# Autodesk Inventor assembly: keel
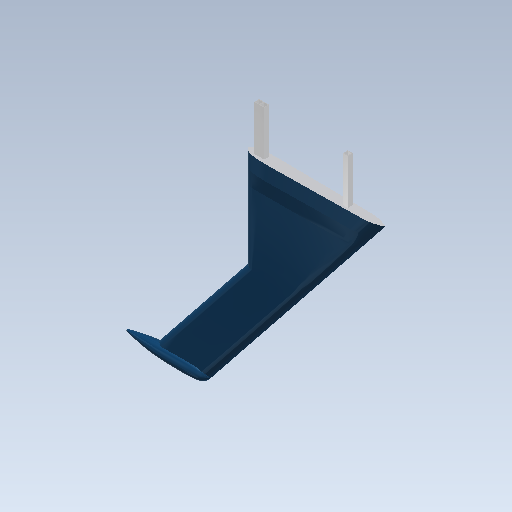
[picture p0: Inventor's stored thumbnail of the model, 512x512]
Saved by Autodesk Inventor 2020 (Build 240168000, 168)
## iProperties
Created: 2017-12-03
Part Number: keel
Document SubType Name: Assembly
Designer: stedrock
Author: stedrock
## Documents named in this file (3)
- C:\Users\jous\Desktop\boat\keel.iam
- C:\Users\jous\Desktop\boat\keel.ipt
- C:\Users\jous\Desktop\boat\keel_bulb.ipt
## Components (2 placed, 2 different names)
1. keel:1 — Mate:1, Mate:2
2. keel_bulb:1 — Mate:1, Mate:2
## Relationships (2: Mate 2)
- Mate:1: keel:1 ↔ keel_bulb:1
- Mate:2: keel:1 ↔ keel_bulb:1
